# Autodesk Inventor assembly: X-Anchor
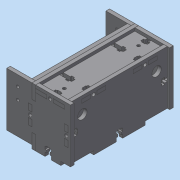
[picture p0: Inventor's stored thumbnail of the model, 180x180]
Saved by Autodesk Inventor 2016 SP1 (Build 200210100, 210)
## iProperties
Created: 2016-01-20
Part Number: X-Anchor
Document SubType Name: Assembly
Designer: Mohamed A.
Author: Mohamed A.
## Documents named in this file (6)
- C:\Users\Mohamed\Documents\inventor\StemCellsPlatform\Laser Cut\X-Anchor\X-Anchor.iam
- C:\Users\Mohamed\Documents\inventor\StemCellsPlatform\Laser Cut\X-Anchor\X-Anchor_Front-Outer.ipt
- C:\Users\Mohamed\Documents\inventor\StemCellsPlatform\Laser Cut\X-Anchor\X-Anchor_Front-Inner.ipt
- C:\Users\Mohamed\Documents\inventor\StemCellsPlatform\Laser Cut\X-Anchor\X-Anchor_Side.ipt
- C:\Users\Mohamed\Documents\inventor\StemCellsPlatform\Laser Cut\X-Anchor\X-Anchor_Back.ipt
- C:\Users\Mohamed\Documents\inventor\StemCellsPlatform\Laser Cut\X-Anchor\X-Anchor_Top.ipt
## Components (6 placed, 5 different names)
1. X-Anchor_Front-Outer:1 — Mate:1, Flush:1, Flush:2, Flush:3, Mate:2, Mate:3, Flush:5, Mate:6, Mate:7, Flush:6, Flush:9, Mate:8
2. X-Anchor_Front-Inner:1 — Mate:1, Flush:1, Flush:2, Mate:9, Flush:10, Mate:10
3. X-Anchor_Side:1 — Flush:3, Mate:2, Mate:3, Flush:4, Mate:4, Mate:5, Flush:7
4. X-Anchor_Back:1 — Flush:4, Mate:4, Mate:5
5. X-Anchor_Side:2 — Flush:5, Mate:6, Mate:7
6. X-Anchor_Top:1 — Flush:6, Flush:7, Flush:9, Mate:8
## Relationships (19: Mate 10, Flush 9)
- Mate:1: X-Anchor_Front-Outer:1 ↔ X-Anchor_Front-Inner:1
- Flush:1: X-Anchor_Front-Outer:1 ↔ X-Anchor_Front-Inner:1
- Flush:2: X-Anchor_Front-Outer:1 ↔ X-Anchor_Front-Inner:1
- Flush:3: X-Anchor_Front-Outer:1 ↔ X-Anchor_Side:1
- Mate:2: X-Anchor_Front-Outer:1 ↔ X-Anchor_Side:1
- Mate:3: X-Anchor_Front-Outer:1 ↔ X-Anchor_Side:1
- Flush:4: X-Anchor_Side:1 ↔ X-Anchor_Back:1
- Mate:4: X-Anchor_Side:1 ↔ X-Anchor_Back:1
- Mate:5: X-Anchor_Side:1 ↔ X-Anchor_Back:1
- Flush:5: X-Anchor_Front-Outer:1 ↔ X-Anchor_Side:2
- Mate:6: X-Anchor_Front-Outer:1 ↔ X-Anchor_Side:2
- Mate:7: X-Anchor_Front-Outer:1 ↔ X-Anchor_Side:2
- Flush:6: X-Anchor_Front-Outer:1 ↔ X-Anchor_Top:1
- Flush:7: X-Anchor_Side:1 ↔ X-Anchor_Top:1
- Flush:9: X-Anchor_Front-Outer:1 ↔ X-Anchor_Top:1
- Mate:8: X-Anchor_Front-Outer:1 ↔ X-Anchor_Top:1
- Mate:9: X-Anchor_Front-Inner:1
- Flush:10: X-Anchor_Front-Inner:1
- Mate:10: X-Anchor_Front-Inner:1
